# Autodesk Inventor assembly: afroesc
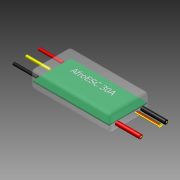
[picture p0: Inventor's stored thumbnail of the model, 180x180]
Saved by Autodesk Inventor 2012 (Build 160160000, 160)
## iProperties
Created: 2014-07-18
Part Number: afroesc
Document SubType Name: Assembly
Designer: Anon
Author: Anon
## Documents named in this file (10)
- D:\Dropbox\Courses\GP\git\dronestructure\electronics\afroesc\afroesc.iam
- D:\Dropbox\Courses\GP\git\dronestructure\electronics\afroesc\esc.ipt
- D:\Dropbox\Courses\GP\git\dronestructure\electronics\afroesc\bigblack.ipt
- D:\Dropbox\Courses\GP\git\dronestructure\electronics\afroesc\bigred.ipt
- D:\Dropbox\Courses\GP\git\dronestructure\electronics\afroesc\yellowlead.ipt
- D:\Dropbox\Courses\GP\git\dronestructure\electronics\afroesc\afro.ipt
- D:\Dropbox\Courses\GP\git\dronestructure\electronics\afroesc\pcb.ipt
- D:\Dropbox\Courses\GP\git\dronestructure\electronics\afroesc\blacklead.ipt
- D:\Dropbox\Courses\GP\git\dronestructure\electronics\afroesc\redlead.ipt
- D:\Dropbox\Courses\GP\git\dronestructure\electronics\afroesc\servoribbon.iam
## Components (9 placed, 9 different names)
1. esc:1 — Flush:1, Flush:2, Flush:3, Mate:2, Mate:3, Mate:11, Mate:12, Mate:13, Mate:14, Mate:17, Flush:6, Mate:19, Flush:20, Mate:20, Mate:21
2. bigblack:1 — Mate:1, Flush:4, Mate:2
3. bigred:1 — Mate:3, Mate:4, Mate:5
4. yellowlead:1 — Mate:16, Mate:17, Flush:6
5. afro:1 — Mate:19, Flush:20, Mate:20
6. pcb:1 — Mate:10, Mate:11, Mate:12
7. blacklead:1 — Mate:14, Mate:15, Flush:5
8. redlead:1 — Mate:13, Mate:18, Flush:7
9. servoribbon:1 [sub-assembly] — Mate:21, Mate:22, Flush:22
## Relationships (28: Mate 18, Flush 10)
- Flush:1 (8 mm): esc:1
- Flush:2 (-8 mm): esc:1
- Mate:1: bigblack:1
- Flush:3 (4 mm): esc:1
- Flush:4: bigblack:1
- Mate:2: esc:1 ↔ bigblack:1
- Mate:3: esc:1 ↔ bigred:1
- Mate:4: bigred:1
- Mate:5: bigred:1
- Mate:10: pcb:1
- Mate:11: esc:1 ↔ pcb:1
- Mate:12: esc:1 ↔ pcb:1
- Mate:13: esc:1 ↔ redlead:1
- Mate:14: esc:1 ↔ blacklead:1
- Mate:15: blacklead:1
- Flush:5: blacklead:1
- Mate:16: yellowlead:1
- Mate:17: esc:1 ↔ yellowlead:1
- Flush:6: esc:1 ↔ yellowlead:1
- Mate:18: redlead:1
- Flush:7: redlead:1
- Mate:19: esc:1 ↔ afro:1
- Flush:20: esc:1 ↔ afro:1
- Mate:20: esc:1 ↔ afro:1
- Mate:21: esc:1 ↔ servoribbon:1
- Mate:22: servoribbon:1
- Flush:21 (-3 mm)
- Flush:22: servoribbon:1
